# Autodesk Inventor assembly: (VEX) Cortex Microcontroller
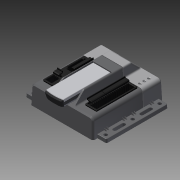
[picture p0: Inventor's stored thumbnail of the model, 180x180]
Saved by Autodesk Inventor 2016 (Build 200138000, 138)
## iProperties
Created: 2011-01-18
Part Number: (VEX) Cortex Microcontroller
Document SubType Name: Assembly
Designer: Jordan
Mass: 136.985 g
Surface Area: 1369.41 cm^2
Volume: 109.727 cm^3
Density: 1.24842 g/cm^3
Translation Standard: STEP AP203
FileName: (VEX) Cortex Microcontroller.iam
PreProcessor: SolidWorks 2010
PostProcessor: Build: 239, Release: 2011 RTM - Date: Wed 02/17/2010
Sent Units: inch
Uncertainty: 1e-05
Author: Jordan
## Documents named in this file (12)
- C:\Users\Jordan\Documents\Robotics\CAD\2015 BNS CAD Library (beta)\Logic\Cortex Microcontroller.iam
- C:\Users\Jordan\Documents\Robotics\CAD\2015 BNS CAD Library (beta)\Logic\Reference Parts\Cortex Microcontroller\276-2194-SWITCH_BUTTON.ipt
- C:\Users\Jordan\Documents\Robotics\CAD\2015 BNS CAD Library (beta)\Logic\Reference Parts\Cortex Microcontroller\276-2194-001 Rev2.ipt
- C:\Users\Jordan\Documents\Robotics\CAD\2015 BNS CAD Library (beta)\Logic\Reference Parts\Cortex Microcontroller\276-2194-LIGHTPIPE.ipt
- C:\Users\Jordan\Documents\Robotics\CAD\2015 BNS CAD Library (beta)\Logic\Reference Parts\Cortex Microcontroller\276-2194-BOTTOM-CASE.ipt
- C:\Users\Jordan\Documents\Robotics\CAD\2015 BNS CAD Library (beta)\Logic\Reference Parts\Cortex Microcontroller\276-2194-SMALL_LOCK_TAB.ipt
- C:\Users\Jordan\Documents\Robotics\CAD\2015 BNS CAD Library (beta)\Logic\Reference Parts\Cortex Microcontroller\276-2194-PWM_LOCK_BUCKET.ipt
- C:\Users\Jordan\Documents\Robotics\CAD\2015 BNS CAD Library (beta)\Logic\Reference Parts\Cortex Microcontroller\276-2194-SHORT_LOCK_TAB.ipt
- C:\Users\Jordan\Documents\Robotics\CAD\2015 BNS CAD Library (beta)\Logic\Reference Parts\Cortex Microcontroller\276-2194-MOTOR_LOCK_BUCKET.ipt
- C:\Users\Jordan\Documents\Robotics\CAD\2015 BNS CAD Library (beta)\Logic\Reference Parts\Cortex Microcontroller\276-2194-2_0_PCB_ASSY_REV2_ANY_ASM.iam
- C:\Users\Jordan\Documents\Robotics\CAD\2015 BNS CAD Library (beta)\Logic\Reference Parts\Cortex Microcontroller\276-2194-LONG_LOCK_TAB.ipt
- C:\Users\Jordan\Documents\Robotics\CAD\2015 BNS CAD Library (beta)\Logic\Reference Parts\VEXnet Microcontrollers\VEXnet Key 2.0.ipt
## Components (13 placed, 11 different names)
1. 276-2194-SWITCH_BUTTON:1
2. 276-2194-001 Rev2:1
3. 276-2194-LIGHTPIPE:1
4. 276-2194-BOTTOM-CASE:1
5. 276-2194-SMALL_LOCK_TAB:1
6. 276-2194-PWM_LOCK_BUCKET:1
7. 276-2194-SHORT_LOCK_TAB:1
8. 276-2194-MOTOR_LOCK_BUCKET:1
9. 276-2194-LIGHTPIPE:2
10. 276-2194-LIGHTPIPE:3
11. 276-2194-2_0_PCB_ASSY_REV2_ANY_ASM:1 [sub-assembly] — Mate:1, Mate:2, Mate:3
12. 276-2194-LONG_LOCK_TAB:1
13. VEXnet Key 2.0:1 — Mate:1, Mate:2, Mate:3
## Relationships (3: Mate 3)
- Mate:1: 276-2194-2_0_PCB_ASSY_REV2_ANY_ASM:1 ↔ VEXnet Key 2.0:1
- Mate:2 (0.2 mm): 276-2194-2_0_PCB_ASSY_REV2_ANY_ASM:1 ↔ VEXnet Key 2.0:1
- Mate:3 (0.3 mm): 276-2194-2_0_PCB_ASSY_REV2_ANY_ASM:1 ↔ VEXnet Key 2.0:1
